# Autodesk Inventor assembly: analog_multiplexer_16pin
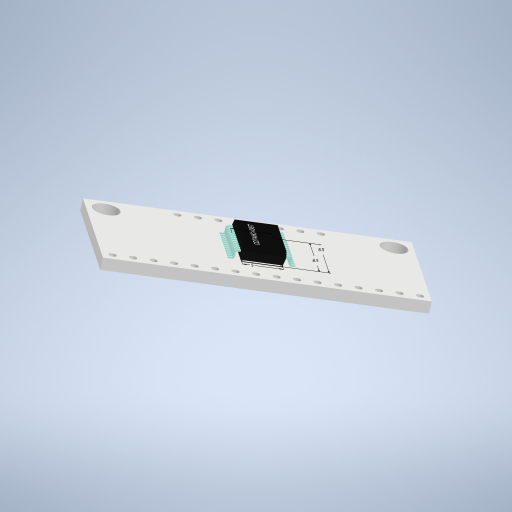
[picture p0: Inventor's stored thumbnail of the model, 512x512]
Saved by Autodesk Inventor 2023.1 (Build 271208000, 208)
## iProperties
Created: 2022-07-25
Part Number: analog_multiplexer_16pin
Document SubType Name: Assembly
Designer: fraaw
Author: fraaw
## Documents named in this file (3)
- C:\Users\fraaw\OneDrive\Desktop\analog_multiplexer_16pin.iam
- C:\Users\fraaw\OneDrive\Desktop\HW-178.ipt
- C:\Users\fraaw\OneDrive\Desktop\CD74HC4067.ipt
## Components (2 placed, 2 different names)
1. HW-178:1 — Rigid:1, Rigid:2
2. CD74HC4067:1 — Rigid:1, Rigid:2
## Relationships (2: WeldJoint 2)
- Rigid:1 [WeldJoint]: HW-178:1 ↔ CD74HC4067:1
- Rigid:2 [WeldJoint]: HW-178:1 ↔ CD74HC4067:1
